# Autodesk Inventor assembly: Cart Frame
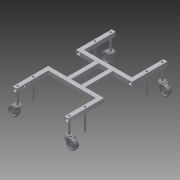
[picture p0: Inventor's stored thumbnail of the model, 180x180]
Saved by Autodesk Inventor 2014 (Build 180170000, 170)
## iProperties
Created: 2014-02-25
Part Number: Cart Frame
Document SubType Name: Assembly
Designer: Nitesh
Mass: 6932.69 g
Surface Area: 5024.38 cm^2
Volume: 872.412 cm^3
Density: 7.94658 g/cm^3
Author: Nitesh
## Documents named in this file (7)
- C:\Users\Nitesh\Desktop\PFP Robot with Cart\Cart Frame.iam
- C:\Users\Nitesh\Desktop\PFP Robot with Cart\Box Cart Center.ipt
- C:\Users\Nitesh\Desktop\PFP Robot with Cart\Box Cart Sides.ipt
- C:\Users\Nitesh\Desktop\PFP Robot with Cart\Box Cart Legs.ipt
- C:\Users\Nitesh\Desktop\PFP Robot with Cart\Caster Wheel Leg.ipt
- C:\Users\Nitesh\Desktop\PFP Robot with Cart\Caster.ipt
- C:\Users\Nitesh\Desktop\PFP Robot with Cart\Bearing Guide.ipt
## Components (20 placed, 6 different names)
1. Box Cart Center:1 — Mate:2, Flush:2, Flush:3, Mate:3, Flush:5
2. Box Cart Center:2 — Mate:1, Flush:1, Flush:4
3. Box Cart Sides:1 — Mate:1, Mate:2, Flush:1, Flush:2, Flush:3, Flush:4, Flush:6, Mate:5, Flush:9, Flush:10, Mate:7, Flush:13, Flush:14
4. Box Cart Sides:2 — Mate:3, Flush:5, Flush:6, Mate:4, Flush:7, Flush:8, Mate:6, Flush:11, Flush:12
5. Box Cart Legs:1 — Mate:4, Flush:7, Flush:8, Flush:15, Mate:8, Mate:20, Flush:19, Angle:1
6. Box Cart Legs:2 — Mate:6, Flush:11, Flush:12, Mate:9, Flush:16, Angle:2, Mate:21, Flush:20
7. Box Cart Legs:3 — Mate:5, Flush:9, Flush:10, Mate:11, Flush:18, Angle:4, Mate:22, Flush:21
8. Box Cart Legs:4 — Mate:7, Flush:13, Flush:14, Mate:10, Flush:17, Angle:3, Mate:23, Flush:22
9. Caster Wheel Leg:1 — Flush:15, Mate:8, Mate:12, Mate:13
10. Caster Wheel Leg:2 — Mate:9, Flush:16, Mate:16, Mate:17
11. Caster Wheel Leg:3 — Mate:11, Flush:18, Mate:14, Mate:15
12. Caster Wheel Leg:4 — Mate:10, Flush:17, Mate:18, Mate:19
13. Caster:1 — Mate:14, Mate:15, Angle:4
14. Caster:2 — Mate:18, Mate:19, Angle:3
15. Caster:3 — Mate:12, Mate:13, Angle:1
16. Caster:4 — Mate:16, Mate:17, Angle:2
17. Bearing Guide:1 — Mate:20, Flush:19
18. Bearing Guide:2 — Mate:21, Flush:20
19. Bearing Guide:3 — Mate:22, Flush:21
20. Bearing Guide:4 — Mate:23, Flush:22
## Relationships (49: Mate 23, Flush 22, Angle 4)
- Mate:1: Box Cart Center:2 ↔ Box Cart Sides:1
- Mate:2: Box Cart Center:1 ↔ Box Cart Sides:1
- Flush:1: Box Cart Center:2 ↔ Box Cart Sides:1
- Flush:2: Box Cart Center:1 ↔ Box Cart Sides:1
- Flush:3 (95.25 mm): Box Cart Center:1 ↔ Box Cart Sides:1
- Flush:4 (95.25 mm): Box Cart Center:2 ↔ Box Cart Sides:1
- Mate:3: Box Cart Center:1 ↔ Box Cart Sides:2
- Flush:5: Box Cart Center:1 ↔ Box Cart Sides:2
- Flush:6: Box Cart Sides:1 ↔ Box Cart Sides:2
- Mate:4: Box Cart Sides:2 ↔ Box Cart Legs:1
- Flush:7: Box Cart Sides:2 ↔ Box Cart Legs:1
- Flush:8: Box Cart Sides:2 ↔ Box Cart Legs:1
- Mate:5: Box Cart Sides:1 ↔ Box Cart Legs:3
- Flush:9: Box Cart Sides:1 ↔ Box Cart Legs:3
- Flush:10: Box Cart Sides:1 ↔ Box Cart Legs:3
- Mate:6: Box Cart Sides:2 ↔ Box Cart Legs:2
- Flush:11: Box Cart Sides:2 ↔ Box Cart Legs:2
- Flush:12: Box Cart Sides:2 ↔ Box Cart Legs:2
- Mate:7: Box Cart Sides:1 ↔ Box Cart Legs:4
- Flush:13: Box Cart Sides:1 ↔ Box Cart Legs:4
- Flush:14: Box Cart Sides:1 ↔ Box Cart Legs:4
- Flush:15: Box Cart Legs:1 ↔ Caster Wheel Leg:1
- Mate:8: Box Cart Legs:1 ↔ Caster Wheel Leg:1
- Mate:9: Box Cart Legs:2 ↔ Caster Wheel Leg:2
- Flush:16: Box Cart Legs:2 ↔ Caster Wheel Leg:2
- Mate:10: Box Cart Legs:4 ↔ Caster Wheel Leg:4
- Flush:17: Box Cart Legs:4 ↔ Caster Wheel Leg:4
- Mate:11: Box Cart Legs:3 ↔ Caster Wheel Leg:3
- Flush:18: Box Cart Legs:3 ↔ Caster Wheel Leg:3
- Mate:12: Caster Wheel Leg:1 ↔ Caster:3
- Mate:13: Caster Wheel Leg:1 ↔ Caster:3
- Mate:14: Caster Wheel Leg:3 ↔ Caster:1
- Mate:15: Caster Wheel Leg:3 ↔ Caster:1
- Mate:16: Caster Wheel Leg:2 ↔ Caster:4
- Mate:17: Caster Wheel Leg:2 ↔ Caster:4
- Mate:18: Caster Wheel Leg:4 ↔ Caster:2
- Mate:19: Caster Wheel Leg:4 ↔ Caster:2
- Mate:20: Box Cart Legs:1 ↔ Bearing Guide:1
- Flush:19: Box Cart Legs:1 ↔ Bearing Guide:1
- Angle:1 (0 deg): Box Cart Legs:1 ↔ Caster:3
- Angle:2 (0 deg): Box Cart Legs:2 ↔ Caster:4
- Angle:3 (0 deg): Box Cart Legs:4 ↔ Caster:2
- Angle:4 (180 deg): Box Cart Legs:3 ↔ Caster:1
- Mate:21: Box Cart Legs:2 ↔ Bearing Guide:2
- Flush:20: Box Cart Legs:2 ↔ Bearing Guide:2
- Mate:22: Box Cart Legs:3 ↔ Bearing Guide:3
- Flush:21: Box Cart Legs:3 ↔ Bearing Guide:3
- Mate:23: Box Cart Legs:4 ↔ Bearing Guide:4
- Flush:22: Box Cart Legs:4 ↔ Bearing Guide:4
